# Autodesk Inventor assembly: Ensamble
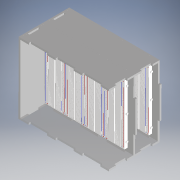
[picture p0: Inventor's stored thumbnail of the model, 180x180]
Saved by Autodesk Inventor 2020 (Build 240168000, 168)
## iProperties
Created: 2020-03-11
Part Number: Ensamble
Document SubType Name: Assembly
Designer: José Javier Estrada
Author: José Javier Estrada
## Documents named in this file (5)
- C:\Users\José Javier Estrada\Downloads\Ensamble.iam
- C:\Users\José Javier Estrada\Downloads\protoboard.ipt
- C:\Users\José Javier Estrada\Downloads\Placa de abajo.ipt
- C:\Users\José Javier Estrada\Downloads\Lateral 1.ipt
- C:\Users\José Javier Estrada\Downloads\Frente.ipt
## Components (13 placed, 4 different names)
1. protoboard:1 — Rigid:1, Rigid:2, Mate:1
2. protoboard:2 — Rigid:1, Rigid:3, Flush:1
3. protoboard:3 — Rigid:3, Flush:2
4. protoboard:4 — Rigid:2
5. Placa de abajo:1 — Mate:1, Flush:1, Flush:2, Rigid:4, Rigid:5, Rigid:10
6. Lateral 1:1 — Rigid:4
7. Lateral 1:2 — Rigid:5, Rigid:9
8. protoboard:5
9. protoboard:6
10. protoboard:7
11. protoboard:8
12. Placa de abajo:2 — Rigid:9
13. Frente:1 — Rigid:10
## Relationships (16: WeldJoint 10, Flush 4, Mate 2)
- Rigid:1 [WeldJoint]: protoboard:1 ↔ protoboard:2
- Rigid:2 [WeldJoint]: protoboard:1 ↔ protoboard:4
- Rigid:3 [WeldJoint]: protoboard:2 ↔ protoboard:3
- Mate:1: protoboard:1 ↔ Placa de abajo:1
- Flush:1 (15 mm): protoboard:2 ↔ Placa de abajo:1
- Flush:2 (10 mm): protoboard:3 ↔ Placa de abajo:1
- Rigid:4 [WeldJoint]: Placa de abajo:1 ↔ Lateral 1:1
- Rigid:5 [WeldJoint]: Placa de abajo:1 ↔ Lateral 1:2
- [WeldJoint]: protoboard:5 ↔ protoboard:6
- [WeldJoint]: protoboard:5 ↔ protoboard:8
- [WeldJoint]: protoboard:6 ↔ protoboard:7
- [Mate]: protoboard:5 ↔ Placa de abajo:2
- [Flush] (15 mm): protoboard:6 ↔ Placa de abajo:2
- [Flush] (10 mm): protoboard:7 ↔ Placa de abajo:2
- Rigid:9 [WeldJoint]: Lateral 1:2 ↔ Placa de abajo:2
- Rigid:10 [WeldJoint]: Placa de abajo:1 ↔ Frente:1
## Named parameters: d8_d0 = 0 mm, d9_d1 = 0 mm, d10_d2 = 0 mm, d11_d3 = 0 mm, d12_d4 = 15 mm, d13_d5 = 10 mm
